# Autodesk Inventor assembly: Lift.00.00.00.00
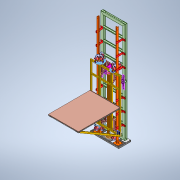
[picture p0: Inventor's stored thumbnail of the model, 180x180]
Saved by Autodesk Inventor 2021 (Build 250183000, 183)
## iProperties
Created: 2020-09-20
Part Number: Lift.00.00.00.00
Document SubType Name: Assembly
Designer: Kostya
_SolveAssemblyDoc: Frame Generator Solve Assembly
_Version: 25.0.0
Author: Kostya
## Documents named in this file (11)
- C:\Lift\Lift.00.00.00.00.iam
- C:\Lift\Lift.00.00.00.08.ipt
- C:\Lift\Lift.00.00.00.00\Frame\Frame 1600626060237.iam
- C:\Lift\Lift.00.00.00.01.ipt
- C:\Lift\Lift.03.00.00.00.iam
- C:\Lift\Lift.01.00.00.00.iam
- C:\Lift\Lift.02.00.00.00.iam
- C:\Lift\Lift.04.00.00.00.iam
- C:\Lift\Lift.00.00.00.07.ipt
- C:\Lift\Lift.00.00.00.02.ipt
- C:\Lift\Lift.00.00.00.07_MIR1.ipt
## Components (24 placed, 10 different names)
1. Lift.00.00.00.08:1 — Совмещение:1, Совмещение:2, Заподлицо:1
2. Frame 1600626060237:1 [sub-assembly] — Совмещение:3, Заподлицо:2, Заподлицо:3, Совмещение:4, Заподлицо:4, Заподлицо:5, Совмещение:5, Заподлицо:6, Совмещение:7, Заподлицо:7, Совмещение:9, Заподлицо:8, Заподлицо:9, Угол:1, Заподлицо:16, Заподлицо:21
3. Lift.00.00.00.01:1 — Совмещение:3, Заподлицо:2, Заподлицо:3, Совмещение:13, Заподлицо:11
4. Lift.00.00.00.01:2 — Совмещение:4, Заподлицо:4, Заподлицо:5, Заподлицо:10
5. Lift.03.00.00.00:1 [sub-assembly] — Совмещение:11, Совмещение:12, Угол:1, Заподлицо:21
6. Lift.01.00.00.00:1 [sub-assembly] — Совмещение:7, Заподлицо:7, Заподлицо:22
7. Lift.01.00.00.00:2 [sub-assembly] — Совмещение:5, Заподлицо:6, Совмещение:22, Совмещение:23, Заподлицо:22, Совмещение:25
8. Lift.02.00.00.00:1 [sub-assembly] — Совмещение:9, Заподлицо:8, Заподлицо:9, Совмещение:11, Совмещение:12
9. Lift.04.00.00.00:1 [sub-assembly] — Совмещение:13, Заподлицо:10, Заподлицо:11, Совмещение:14, Заподлицо:12, Заподлицо:13, Совмещение:19, Совмещение:24, Заподлицо:24
10. Lift.04.00.00.00:2 [sub-assembly] — Совмещение:14, Заподлицо:12, Заподлицо:13, Заподлицо:17, Заподлицо:18, Совмещение:20, Заподлицо:19, Заподлицо:20, Совмещение:21, Заподлицо:23
11. Lift.00.00.00.02:1 — Совмещение:19, Заподлицо:17, Заподлицо:18
12. Lift.00.00.00.02:2 — Совмещение:20, Заподлицо:19, Заподлицо:20
13. Lift.00.00.00.07_MIR1:1
14. Lift.00.00.00.07_MIR1:2
15. Lift.00.00.00.07_MIR1:3
16. Lift.00.00.00.07_MIR1:4
17. Lift.00.00.00.07_MIR1:5
18. Lift.00.00.00.07_MIR1:6
19. Lift.00.00.00.07:1 — Совмещение:21, Совмещение:22, Совмещение:23, Заподлицо:23
20. Lift.00.00.00.07:5
21. Lift.00.00.00.07:6
22. Lift.00.00.00.07:4 — Совмещение:24, Совмещение:25, Заподлицо:24
23. Lift.00.00.00.07:7
24. Lift.00.00.00.07:8
## Component patterns: (3 elements, first: Lift.00.00.00.07:1), (3 elements, first: Lift.00.00.00.07:4)
## Relationships (41: Flush 22, Mate 18, Angle 1)
- Совмещение:1 [Mate]: Lift.00.00.00.08:1
- Совмещение:2 [Mate]: Lift.00.00.00.08:1
- Заподлицо:1 [Flush]: Lift.00.00.00.08:1
- Совмещение:3 [Mate]: Frame 1600626060237:1 ↔ Lift.00.00.00.01:1
- Заподлицо:2 [Flush]: Frame 1600626060237:1 ↔ Lift.00.00.00.01:1
- Заподлицо:3 [Flush]: Frame 1600626060237:1 ↔ Lift.00.00.00.01:1
- Совмещение:4 [Mate]: Frame 1600626060237:1 ↔ Lift.00.00.00.01:2
- Заподлицо:4 [Flush]: Frame 1600626060237:1 ↔ Lift.00.00.00.01:2
- Заподлицо:5 [Flush]: Frame 1600626060237:1 ↔ Lift.00.00.00.01:2
- Совмещение:5 [Mate]: Frame 1600626060237:1 ↔ Lift.01.00.00.00:2
- Заподлицо:6 [Flush]: Frame 1600626060237:1 ↔ Lift.01.00.00.00:2
- Совмещение:7 [Mate]: Frame 1600626060237:1 ↔ Lift.01.00.00.00:1
- Заподлицо:7 [Flush]: Frame 1600626060237:1 ↔ Lift.01.00.00.00:1
- Совмещение:9 [Mate]: Frame 1600626060237:1 ↔ Lift.02.00.00.00:1
- Заподлицо:8 [Flush] (35 mm): Frame 1600626060237:1 ↔ Lift.02.00.00.00:1
- Заподлицо:9 [Flush]: Frame 1600626060237:1 ↔ Lift.02.00.00.00:1
- Совмещение:11 [Mate] (30 mm): Lift.03.00.00.00:1 ↔ Lift.02.00.00.00:1
- Совмещение:12 [Mate]: Lift.03.00.00.00:1 ↔ Lift.02.00.00.00:1
- Угол:1 [Angle] (0 deg): Frame 1600626060237:1 ↔ Lift.03.00.00.00:1
- Совмещение:13 [Mate]: Lift.00.00.00.01:1 ↔ Lift.04.00.00.00:1
- Заподлицо:10 [Flush] (32.5 mm): Lift.00.00.00.01:2 ↔ Lift.04.00.00.00:1
- Заподлицо:11 [Flush] (80 mm): Lift.00.00.00.01:1 ↔ Lift.04.00.00.00:1
- Совмещение:14 [Mate]: Lift.04.00.00.00:1 ↔ Lift.04.00.00.00:2
- Заподлицо:12 [Flush]: Lift.04.00.00.00:1 ↔ Lift.04.00.00.00:2
- Заподлицо:13 [Flush]: Lift.04.00.00.00:1 ↔ Lift.04.00.00.00:2
- Заподлицо:16 [Flush] (-857 mm): Frame 1600626060237:1
- Совмещение:19 [Mate]: Lift.04.00.00.00:1 ↔ Lift.00.00.00.02:1
- Заподлицо:17 [Flush]: Lift.04.00.00.00:2 ↔ Lift.00.00.00.02:1
- Заподлицо:18 [Flush] (-2635 mm): Lift.04.00.00.00:2 ↔ Lift.00.00.00.02:1
- Совмещение:20 [Mate]: Lift.04.00.00.00:2 ↔ Lift.00.00.00.02:2
- Заподлицо:19 [Flush]: Lift.04.00.00.00:2 ↔ Lift.00.00.00.02:2
- Заподлицо:20 [Flush] (2635 mm): Lift.04.00.00.00:2 ↔ Lift.00.00.00.02:2
- Заподлицо:21 [Flush]: Frame 1600626060237:1 ↔ Lift.03.00.00.00:1
- Совмещение:21 [Mate]: Lift.04.00.00.00:2 ↔ Lift.00.00.00.07:1
- Совмещение:22 [Mate]: Lift.01.00.00.00:2 ↔ Lift.00.00.00.07:1
- Совмещение:23 [Mate]: Lift.01.00.00.00:2 ↔ Lift.00.00.00.07:1
- Заподлицо:22 [Flush]: Lift.01.00.00.00:1 ↔ Lift.01.00.00.00:2
- Заподлицо:23 [Flush]: Lift.04.00.00.00:2 ↔ Lift.00.00.00.07:1
- Совмещение:24 [Mate]: Lift.04.00.00.00:1 ↔ Lift.00.00.00.07:4
- Совмещение:25 [Mate]: Lift.01.00.00.00:2 ↔ Lift.00.00.00.07:4
- Заподлицо:24 [Flush]: Lift.04.00.00.00:1 ↔ Lift.00.00.00.07:4
